# Autodesk Inventor assembly: RAMPS14
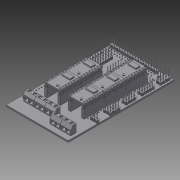
[picture p0: Inventor's stored thumbnail of the model, 180x180]
Saved by Autodesk Inventor 2014 (Build 180170000, 170)
## iProperties
Created: 2014-11-10
Part Number: RAMPS14
Document SubType Name: Assembly
Designer: ThatOtherGuy
Author: ThatOtherGuy
## Documents named in this file (14)
- C:\Users\ThatOtherGuy\Documents\Inventor\KosselCNC1515\Electronics\RAMPS14.iam
- C:\Users\ThatOtherGuy\Documents\Inventor\KosselCNC1515\Electronics\RAMPS14.ipt
- C:\Users\ThatOtherGuy\Documents\Inventor\Content Center Files\R2014\en-US\Header_Male\Header_Male_1x10.ipt
- C:\Users\ThatOtherGuy\Documents\Inventor\Content Center Files\R2014\en-US\Header_Male\Header_Male_1x8.ipt
- C:\Users\ThatOtherGuy\Documents\Inventor\Content Center Files\R2014\en-US\Header_Male\Header_Male_2x18.ipt
- C:\Users\ThatOtherGuy\Documents\Inventor\Content Center Files\R2014\en-US\Header_Male\Header_Male_1x18.ipt
- C:\Users\ThatOtherGuy\Documents\Inventor\Content Center Files\R2014\en-US\Header_Male\Header_Male_2x4.ipt
- C:\Users\ThatOtherGuy\Documents\Inventor\Content Center Files\R2014\en-US\Header_Male\Header_Male_2x5.ipt
- C:\Users\ThatOtherGuy\Documents\Inventor\Content Center Files\R2014\en-US\Header_Male\Header_Male_1x3.ipt
- C:\Users\ThatOtherGuy\Documents\Inventor\Content Center Files\R2014\en-US\Header_Male\Header_Male_2x3.ipt
- C:\Users\ThatOtherGuy\Documents\Inventor\Content Center Files\R2014\en-US\Header_Female\Header_Female_1x8.ipt
- C:\Users\ThatOtherGuy\Documents\Inventor\KosselCNC1515\Electronics\DRV8825_Pololu_Carrier.ipt
- C:\Users\ThatOtherGuy\Documents\Inventor\Content Center Files\R2014\en-US\Header_Male\Header_Male_1x4.ipt
- C:\Users\ThatOtherGuy\Documents\Inventor\Content Center Files\R2014\en-US\Header_Male\Header_Male_1x6.ipt
## Components (45 placed, 13 different names)
1. RAMPS1.4:1 — Insert:1, Insert:2, Insert:3, Insert:4, Insert:5, Insert:6, Insert:7, Insert:8, Insert:9, Insert:10, Insert:11, Insert:12, Insert:13, Insert:14, Insert:59, Insert:60, Insert:61, Insert:62, Insert:63, Insert:64, Insert:65, Insert:66, Insert:67, Insert:68, Insert:69, Insert:70, Insert:71, Insert:72, Insert:73, Insert:74, Insert:75, Insert:76, Insert:77, Insert:78, Insert:79, Insert:80, Insert:81, Insert:82, Insert:83, Insert:84, Insert:85, Insert:86, Insert:87, Insert:88, Insert:89, Insert:90, Insert:91, Insert:92, Insert:93, Insert:94, Insert:95, Insert:96, Insert:97, Insert:98, Insert:99, Insert:100, Insert:101, Insert:102, Insert:103, Insert:104, Insert:105, Insert:106, Insert:107, Insert:108, Insert:109, Insert:110, Insert:111, Insert:112, Insert:113, Insert:114, Insert:115, Insert:116, Insert:117, Insert:118, Insert:119, Insert:120, Insert:121, Insert:122
2. DRV8825_Pololu_Carrier:2 — Insert:123, Insert:124
3. DRV8825_Pololu_Carrier:3 — Insert:125, Insert:126
4. DRV8825_Pololu_Carrier:4 — Insert:127, Insert:128
5. DRV8825_Pololu_Carrier:5 — Insert:129, Insert:130
6. Header_Male 1-10:1 — Insert:1, Insert:2
7. Header_Male 1-8:1 — Insert:3, Insert:4
8. Header_Male 1-8:2 — Insert:5, Insert:6
9. Header_Male 1-8:3 — Insert:7, Insert:8
10. Header_Male 1-8:4 — Insert:9, Insert:10
11. Header_Male 1-8:5 — Insert:11, Insert:12
12. Header_Male 2-18:1 — Insert:13, Insert:14
13. Header_Female 1-8:1 — Insert:75, Insert:76, Insert:127
14. Header_Female 1-8:2 — Insert:77, Insert:78, Insert:129
15. Header_Female 1-8:3 — Insert:73, Insert:74, Insert:128
16. Header_Female 1-8:4 — Insert:79, Insert:84, Insert:130
17. Header_Female 1-8:5 — Insert:49, Insert:80, Insert:81
18. Header_Female 1-8:6 — Insert:89, Insert:90, Insert:124
19. Header_Female 1-8:7 — Insert:86, Insert:88, Insert:126
20. Header_Female 1-8:8 — Insert:50, Insert:82, Insert:83
21. Header_Female 1-8:9 — Insert:91, Insert:92, Insert:123
22. Header_Female 1-8:10 — Insert:85, Insert:87, Insert:125
23. Header_Male 1-18:1 — Insert:71, Insert:72
24. Header_Male 2-4:1 — Insert:69, Insert:70
25. Header_Male 2-4:2 — Insert:65, Insert:66
26. Header_Male 2-5:1 — Insert:67, Insert:68
27. Header_Male 1-3:1 — Insert:59, Insert:60
28. Header_Male 2-3:1 — Insert:61, Insert:62
29. Header_Male 2-3:2 — Insert:63, Insert:64
30. Header_Male 1-4:1 — Insert:109, Insert:110
31. Header_Male 1-4:2 — Insert:111, Insert:112
32. Header_Male 1-4:3 — Insert:113, Insert:114
33. Header_Male 1-4:4 — Insert:115, Insert:116
34. Header_Male 2-4:3 — Insert:117, Insert:118
35. DRV8825_Pololu_Carrier:1 — Insert:49, Insert:50
36. Header_Male 2-3:3 — Insert:101, Insert:102
37. Header_Male 2-3:4 — Insert:99, Insert:100
38. Header_Male 2-3:5 — Insert:93, Insert:94
39. Header_Male 2-3:6 — Insert:95, Insert:96
40. Header_Male 2-3:7 — Insert:97, Insert:98
41. Header_Male 1-6:1 — Insert:121, Insert:122
42. Header_Male 1-4:5 — Insert:119, Insert:120
43. Header_Male 2-3:8 — Insert:103, Insert:104
44. Header_Male 2-3:9 — Insert:105, Insert:106
45. Header_Male 2-3:10 — Insert:107, Insert:108
## Relationships (88: Insert 88)
- Insert:1: RAMPS1.4:1 ↔ Header_Male 1-10:1
- Insert:2: RAMPS1.4:1 ↔ Header_Male 1-10:1
- Insert:3: RAMPS1.4:1 ↔ Header_Male 1-8:1
- Insert:4: RAMPS1.4:1 ↔ Header_Male 1-8:1
- Insert:5: RAMPS1.4:1 ↔ Header_Male 1-8:2
- Insert:6: RAMPS1.4:1 ↔ Header_Male 1-8:2
- Insert:7: RAMPS1.4:1 ↔ Header_Male 1-8:3
- Insert:8: RAMPS1.4:1 ↔ Header_Male 1-8:3
- Insert:9: RAMPS1.4:1 ↔ Header_Male 1-8:4
- Insert:10: RAMPS1.4:1 ↔ Header_Male 1-8:4
- Insert:11: RAMPS1.4:1 ↔ Header_Male 1-8:5
- Insert:12: RAMPS1.4:1 ↔ Header_Male 1-8:5
- Insert:13: RAMPS1.4:1 ↔ Header_Male 2-18:1
- Insert:14: RAMPS1.4:1 ↔ Header_Male 2-18:1
- Insert:49 (0.5 mm): Header_Female 1-8:5 ↔ DRV8825_Pololu_Carrier:1
- Insert:50 (0.5 mm): Header_Female 1-8:8 ↔ DRV8825_Pololu_Carrier:1
- Insert:59: RAMPS1.4:1 ↔ Header_Male 1-3:1
- Insert:60: RAMPS1.4:1 ↔ Header_Male 1-3:1
- Insert:61: RAMPS1.4:1 ↔ Header_Male 2-3:1
- Insert:62: RAMPS1.4:1 ↔ Header_Male 2-3:1
- Insert:63: RAMPS1.4:1 ↔ Header_Male 2-3:2
- Insert:64: RAMPS1.4:1 ↔ Header_Male 2-3:2
- Insert:65: RAMPS1.4:1 ↔ Header_Male 2-4:2
- Insert:66: RAMPS1.4:1 ↔ Header_Male 2-4:2
- Insert:67: RAMPS1.4:1 ↔ Header_Male 2-5:1
- Insert:68: RAMPS1.4:1 ↔ Header_Male 2-5:1
- Insert:69: RAMPS1.4:1 ↔ Header_Male 2-4:1
- Insert:70: RAMPS1.4:1 ↔ Header_Male 2-4:1
- Insert:71: RAMPS1.4:1 ↔ Header_Male 1-18:1
- Insert:72: RAMPS1.4:1 ↔ Header_Male 1-18:1
- Insert:73: RAMPS1.4:1 ↔ Header_Female 1-8:3
- Insert:74: RAMPS1.4:1 ↔ Header_Female 1-8:3
- Insert:75: RAMPS1.4:1 ↔ Header_Female 1-8:1
- Insert:76: RAMPS1.4:1 ↔ Header_Female 1-8:1
- Insert:77: RAMPS1.4:1 ↔ Header_Female 1-8:2
- Insert:78: RAMPS1.4:1 ↔ Header_Female 1-8:2
- Insert:79: RAMPS1.4:1 ↔ Header_Female 1-8:4
- Insert:80: RAMPS1.4:1 ↔ Header_Female 1-8:5
- Insert:81: RAMPS1.4:1 ↔ Header_Female 1-8:5
- Insert:82: RAMPS1.4:1 ↔ Header_Female 1-8:8
- Insert:83: RAMPS1.4:1 ↔ Header_Female 1-8:8
- Insert:84: RAMPS1.4:1 ↔ Header_Female 1-8:4
- Insert:85: RAMPS1.4:1 ↔ Header_Female 1-8:10
- Insert:86: RAMPS1.4:1 ↔ Header_Female 1-8:7
- Insert:87: RAMPS1.4:1 ↔ Header_Female 1-8:10
- Insert:88: RAMPS1.4:1 ↔ Header_Female 1-8:7
- Insert:89: RAMPS1.4:1 ↔ Header_Female 1-8:6
- Insert:90: RAMPS1.4:1 ↔ Header_Female 1-8:6
- Insert:91: RAMPS1.4:1 ↔ Header_Female 1-8:9
- Insert:92: RAMPS1.4:1 ↔ Header_Female 1-8:9
- Insert:93: RAMPS1.4:1 ↔ Header_Male 2-3:5
- Insert:94: RAMPS1.4:1 ↔ Header_Male 2-3:5
- Insert:95: RAMPS1.4:1 ↔ Header_Male 2-3:6
- Insert:96: RAMPS1.4:1 ↔ Header_Male 2-3:6
- Insert:97: RAMPS1.4:1 ↔ Header_Male 2-3:7
- Insert:98: RAMPS1.4:1 ↔ Header_Male 2-3:7
- Insert:99: RAMPS1.4:1 ↔ Header_Male 2-3:4
- Insert:100: RAMPS1.4:1 ↔ Header_Male 2-3:4
- Insert:101: RAMPS1.4:1 ↔ Header_Male 2-3:3
- Insert:102: RAMPS1.4:1 ↔ Header_Male 2-3:3
- Insert:103: RAMPS1.4:1 ↔ Header_Male 2-3:8
- Insert:104: RAMPS1.4:1 ↔ Header_Male 2-3:8
- Insert:105: RAMPS1.4:1 ↔ Header_Male 2-3:9
- Insert:106: RAMPS1.4:1 ↔ Header_Male 2-3:9
- Insert:107: RAMPS1.4:1 ↔ Header_Male 2-3:10
- Insert:108: RAMPS1.4:1 ↔ Header_Male 2-3:10
- Insert:109: RAMPS1.4:1 ↔ Header_Male 1-4:1
- Insert:110: RAMPS1.4:1 ↔ Header_Male 1-4:1
- Insert:111: RAMPS1.4:1 ↔ Header_Male 1-4:2
- Insert:112: RAMPS1.4:1 ↔ Header_Male 1-4:2
- Insert:113: RAMPS1.4:1 ↔ Header_Male 1-4:3
- Insert:114: RAMPS1.4:1 ↔ Header_Male 1-4:3
- Insert:115: RAMPS1.4:1 ↔ Header_Male 1-4:4
- Insert:116: RAMPS1.4:1 ↔ Header_Male 1-4:4
- Insert:117: RAMPS1.4:1 ↔ Header_Male 2-4:3
- Insert:118: RAMPS1.4:1 ↔ Header_Male 2-4:3
- Insert:119: RAMPS1.4:1 ↔ Header_Male 1-4:5
- Insert:120: RAMPS1.4:1 ↔ Header_Male 1-4:5
- Insert:121: RAMPS1.4:1 ↔ Header_Male 1-6:1
- Insert:122: RAMPS1.4:1 ↔ Header_Male 1-6:1
- Insert:123 (0.5 mm): DRV8825_Pololu_Carrier:2 ↔ Header_Female 1-8:9
- Insert:124 (0.5 mm): DRV8825_Pololu_Carrier:2 ↔ Header_Female 1-8:6
- Insert:125 (0.5 mm): DRV8825_Pololu_Carrier:3 ↔ Header_Female 1-8:10
- Insert:126 (0.5 mm): DRV8825_Pololu_Carrier:3 ↔ Header_Female 1-8:7
- Insert:127 (0.5 mm): DRV8825_Pololu_Carrier:4 ↔ Header_Female 1-8:1
- Insert:128 (0.5 mm): DRV8825_Pololu_Carrier:4 ↔ Header_Female 1-8:3
- Insert:129 (0.5 mm): DRV8825_Pololu_Carrier:5 ↔ Header_Female 1-8:2
- Insert:130 (0.5 mm): DRV8825_Pololu_Carrier:5 ↔ Header_Female 1-8:4
